# Autodesk Inventor assembly: motor_1613_2
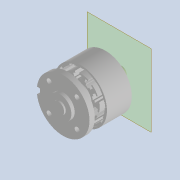
[picture p0: Inventor's stored thumbnail of the model, 180x180]
Saved by Autodesk Inventor 2020 (Build 240168000, 168)
## iProperties
Created: 2022-01-09
Part Number: motor_1613_2
Document SubType Name: Assembly
Designer: Shuang Peng
Author: Shuang Peng
## Documents named in this file (3)
- D:\projects-3\soft module robot\hardware\diff module 3\motor_1613_2.iam
- D:\projects-3\soft module robot\hardware\diff module 3\motor_1613_inner.ipt
- D:\projects-3\soft module robot\hardware\diff module 3\motor_1613_outer.ipt
## Components (2 placed, 2 different names)
1. motor_1613_inner:1 — Insert:1, Flush:1, Angle:1
2. motor_1613_outer:1 — Insert:1, Angle:1
## Relationships (3: Insert 1, Flush 1, Angle 1)
- Insert:1 (-4.3 mm): motor_1613_inner:1 ↔ motor_1613_outer:1
- Flush:1: motor_1613_inner:1
- Angle:1 (0 deg): motor_1613_inner:1 ↔ motor_1613_outer:1
